# Autodesk Inventor assembly: Magazine assebmly
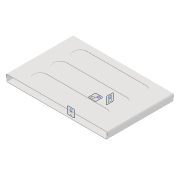
[picture p0: Inventor's stored thumbnail of the model, 180x180]
Saved by Autodesk Inventor 2021 (Build 250183000, 183)
## iProperties
Created: 2020-10-29
Part Number: Magazine assebmly
Document SubType Name: Assembly
Designer: Alfred Brauner
Author: Alfred Brauner
## Documents named in this file (4)
- C:\Users\Alfred Brauner\Documents\Inventor\STOMPA\Magazine assebmly.iam
- C:\Users\Alfred Brauner\Documents\Inventor\STOMPA\Magazine bottom.ipt
- C:\Users\Alfred Brauner\Documents\Inventor\STOMPA\Magazine top.ipt
- C:\Users\Alfred Brauner\Documents\Inventor\STOMPA\Hanging bracket female.ipt
## Components (3 placed, 3 different names)
1. Magazine bottom:1 — Mate:1, Flush:1, Mate:2, Mate:3, Flush:2, Flush:3
2. Magazine top:1 — Mate:1, Flush:1, Mate:2
3. Hanging bracket female:1 — Mate:3, Flush:2, Flush:3
## Relationships (6: Mate 3, Flush 3)
- Mate:1: Magazine bottom:1 ↔ Magazine top:1
- Flush:1: Magazine bottom:1 ↔ Magazine top:1
- Mate:2: Magazine bottom:1 ↔ Magazine top:1
- Mate:3: Magazine bottom:1 ↔ Hanging bracket female:1
- Flush:2 (20 mm): Magazine bottom:1 ↔ Hanging bracket female:1
- Flush:3 (109.5 mm): Magazine bottom:1 ↔ Hanging bracket female:1
